# Autodesk Inventor assembly: centre wing
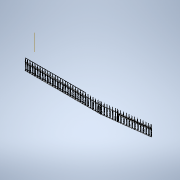
[picture p0: Inventor's stored thumbnail of the model, 180x180]
Saved by Autodesk Inventor 2022 (Build 260153000, 153)
## iProperties
Created: 2021-03-09
Part Number: centre wing
Document SubType Name: Assembly
Designer: Ferdinand Hubbard
Author: Ferdinand Hubbard
## Documents named in this file (3)
- C:\Users\Ferdinand Hubbard\Desktop\solarplane\cad\full wing.iam
- C:\Users\Ferdinand Hubbard\Desktop\solarplane\cad\centre wing section.iam
- C:\Users\Ferdinand Hubbard\Desktop\solarplane\cad\right wing section.iam
## Components (2 placed, 2 different names)
1. centre wing section:1 [sub-assembly] — Mate:1, Mate:2, Mate:3, Mate:4
2. right wing section:1 [sub-assembly] — Mate:1, Mate:2, Mate:3, Mate:4
## Relationships (4: Mate 4)
- Mate:1: centre wing section:1 ↔ right wing section:1
- Mate:2: centre wing section:1 ↔ right wing section:1
- Mate:3: centre wing section:1 ↔ right wing section:1
- Mate:4: centre wing section:1 ↔ right wing section:1
